# Autodesk Inventor assembly: Overall Inside Assembly
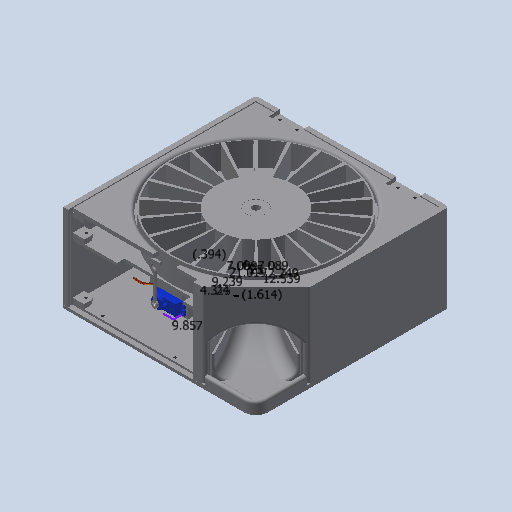
[picture p0: Inventor's stored thumbnail of the model, 512x512]
Saved by Autodesk Inventor 2022 (Build 260153000, 153)
## iProperties
Created: 2023-03-06
Part Number: Overall Inside Assembly
Document SubType Name: Assembly
Designer: zarek
Author: zarek
## Documents named in this file (5)
- C:\Users\zarek\OneDrive\Desktop\Random New Stuff\SPB\Overall Inside Assembly.iam
- C:\Users\zarek\OneDrive\Desktop\Random New Stuff\SPB\Inside Mechanisms.iam
- C:\Users\zarek\OneDrive\Desktop\Random New Stuff\SPB\Box Walls + Top Lid.iam
- C:\Users\zarek\OneDrive\Desktop\Random New Stuff\SPB\Rotational_Piece_2.iam
- C:\Users\zarek\OneDrive\Desktop\Random New Stuff\SPB\Ball_Bearing_Mock_8_22_7mm.ipt
## Components (4 placed, 4 different names)
1. Inside Mechanisms:1 [sub-assembly] — Rigid:1, Rotational:1
2. Box Walls + Top Lid:1 [sub-assembly] — Rotational:1
3. Rotational_Piece_2:1 [sub-assembly] — Rigid:1, Rotational:2
4. Ball_Bearing_Mock_8_22_7mm:1 — Rotational:2
## Relationships (3: RevoluteJoint 2, WeldJoint 1)
- Rigid:1 [WeldJoint]: Inside Mechanisms:1 ↔ Rotational_Piece_2:1
- Rotational:1 [RevoluteJoint]: Inside Mechanisms:1 ↔ Box Walls + Top Lid:1
- Rotational:2 [RevoluteJoint]: Rotational_Piece_2:1 ↔ Ball_Bearing_Mock_8_22_7mm:1
